# Autodesk Inventor assembly: SDS MK4i Swerve Module, NEOs
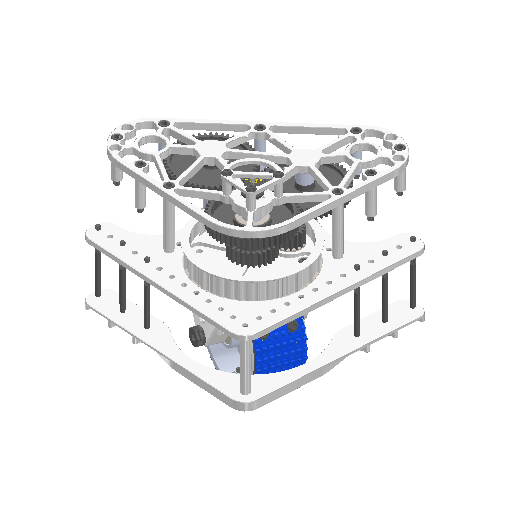
[picture p0: Inventor's stored thumbnail of the model, 512x512]
Saved by Autodesk Inventor 2023 (Build 270158000, 158)
## iProperties
Created: 2023-03-28
Part Number: SDS MK4i Swerve Module, NEOs
Document SubType Name: Assembly
Designer: jackc
Sending System: SOLIDWORKS 2021-2021301
MC: AMD64
MC_MODEL: Intel64 Family 6 Model 158 Stepping 10, GenuineIntel
OS: Windows_NT
FRU: Parasolid Version 32.1, build 255,  1- 1-2021
FORMAT: text
GUISE: transmit
KEY: SDS MK4i Swerve Module, NEOs
FILE: SDS MK4i Swerve Module, NEOs.x_t
DATE: Sun Dec  5 23:34:20 2021
Author: jackc
## Documents named in this file (54)
- J:\My Drive\1939\2_Design\2023-2024\Parts\Swerve\SDS MK4i Swerve Module, unpopulated.iam
- J:\My Drive\1939\2_Design\2023-2024\Parts\Swerve\Screw, 10-32 X .25, Button, 91255A261.ipt
- J:\My Drive\1939\2_Design\2023-2024\Parts\Swerve\Screw, Shoulder, .375 X 2.5, 5_16-18, 91259A634.ipt
- J:\My Drive\1939\2_Design\2023-2024\Parts\Swerve\Screw, .25-20 X 1 Socket, 91251A542.ipt
- J:\My Drive\1939\2_Design\2023-2024\Parts\Swerve\Screw, .25-20 X .625, 91251A539.ipt
- J:\My Drive\1939\2_Design\2023-2024\Parts\Swerve\Screw, 12-24 X .625, Flat, 91253A282.ipt
- J:\My Drive\1939\2_Design\2023-2024\Parts\Swerve\Screw, 10-32 X 1.375, 90044A202.ipt
- J:\My Drive\1939\2_Design\2023-2024\Parts\Swerve\Screw, 10-32 X 2.25, 91251A354.ipt
- J:\My Drive\1939\2_Design\2023-2024\Parts\Swerve\Screw, 8-32 X 2.5, 91251A207.ipt
- J:\My Drive\1939\2_Design\2023-2024\Parts\Swerve\Screw, 8-32 X .875, Button, 91255A166.ipt
- J:\My Drive\1939\2_Design\2023-2024\Parts\Swerve\Screw, 8-32 X .875, Button, 91255A166_1.ipt
- J:\My Drive\1939\2_Design\2023-2024\Parts\Swerve\Shim, 8mm ID X 14mm OD X .5mm Thick, 98055A115.ipt
- J:\My Drive\1939\2_Design\2023-2024\Parts\Swerve\Bearing, 6802.ipt
- J:\My Drive\1939\2_Design\2023-2024\Parts\Swerve\Bearing, R6ZZ.ipt
- J:\My Drive\1939\2_Design\2023-2024\Parts\Swerve\Bearing, R8ZZ.ipt
- J:\My Drive\1939\2_Design\2023-2024\Parts\Swerve\Bearing, 688.ipt
- J:\My Drive\1939\2_Design\2023-2024\Parts\Swerve\Bearing, .375 ThunderHex, Flanged, 217-5829.ipt
- J:\My Drive\1939\2_Design\2023-2024\Parts\Swerve\Bevel Gear, 1545.ipt
- J:\My Drive\1939\2_Design\2023-2024\Parts\Swerve\Bearing, R188ZZ, 217-3489.ipt
- J:\My Drive\1939\2_Design\2023-2024\Parts\Swerve\Bearing, A035XPO_SA035XPO.ipt
- J:\My Drive\1939\2_Design\2023-2024\Parts\Swerve\Double Gear, 20DP, 27T, 50T.ipt
- J:\My Drive\1939\2_Design\2023-2024\Parts\Swerve\Gear, 50T, 20DP, .375Hex.ipt
- J:\My Drive\1939\2_Design\2023-2024\Parts\Swerve\Bevel Gear, 4515.ipt
- J:\My Drive\1939\2_Design\2023-2024\Parts\Swerve\Gear, 20DP, 16T, .375Hex, 217-5451.ipt
- J:\My Drive\1939\2_Design\2023-2024\Parts\Swerve\MK4i Steering Shaft Tall(Default).ipt
- J:\My Drive\1939\2_Design\2023-2024\Parts\Swerve\MK4i Steering Shaft Tall(Default)_1.ipt
- J:\My Drive\1939\2_Design\2023-2024\Parts\Swerve\MK4i Steering Shaft Spacer.ipt
- J:\My Drive\1939\2_Design\2023-2024\Parts\Swerve\MK4 Intermediate Shaft(Default).ipt
- J:\My Drive\1939\2_Design\2023-2024\Parts\Swerve\MK3 Center Column(Default).ipt
- J:\My Drive\1939\2_Design\2023-2024\Parts\Swerve\MK4i Shaft, Drive Idler.ipt
- J:\My Drive\1939\2_Design\2023-2024\Parts\Swerve\CANcoder Assembly.iam
- J:\My Drive\1939\2_Design\2023-2024\Parts\Swerve\magnet.ipt
- J:\My Drive\1939\2_Design\2023-2024\Parts\Swerve\MK4i Master Part(NEO Config).ipt
- J:\My Drive\1939\2_Design\2023-2024\Parts\Swerve\MK4i Master Part(NEO Config)_1.ipt
- J:\My Drive\1939\2_Design\2023-2024\Parts\Swerve\MK4i Master Part(NEO Config)_2.ipt
- J:\My Drive\1939\2_Design\2023-2024\Parts\Swerve\MK4i Master Part(NEO Config)_3.ipt
- J:\My Drive\1939\2_Design\2023-2024\Parts\Swerve\MK4i Master Part(NEO Config)_4.ipt
- J:\My Drive\1939\2_Design\2023-2024\Parts\Swerve\MK4i Master Part(NEO Config)_5.ipt
- J:\My Drive\1939\2_Design\2023-2024\Parts\Swerve\MK4i Master Part(NEO Config)_6.ipt
- J:\My Drive\1939\2_Design\2023-2024\Parts\Swerve\MK4i Master Part(NEO Config)_7.ipt
- J:\My Drive\1939\2_Design\2023-2024\Parts\Swerve\MK4i Master Part(NEO Config)_8.ipt
- J:\My Drive\1939\2_Design\2023-2024\Parts\Swerve\MK4i Master Part(NEO Config)_9.ipt
- J:\My Drive\1939\2_Design\2023-2024\Parts\Swerve\MK4i Master Part(NEO Config)_10.ipt
- J:\My Drive\1939\2_Design\2023-2024\Parts\Swerve\MK4i Master Part(NEO Config)_11.ipt
- J:\My Drive\1939\2_Design\2023-2024\Parts\Swerve\MK4i Master Part(NEO Config)_12.ipt
- J:\My Drive\1939\2_Design\2023-2024\Parts\Swerve\MK4i Master Part(NEO Config)_13.ipt
- J:\My Drive\1939\2_Design\2023-2024\Parts\Swerve\MK4i Master Part(NEO Config)_14.ipt
- J:\My Drive\1939\2_Design\2023-2024\Parts\Swerve\MK4i Master Part(NEO Config)_15.ipt
- J:\My Drive\1939\2_Design\2023-2024\Parts\Swerve\MK4i Master Part(NEO Config)_16.ipt
- J:\My Drive\1939\2_Design\2023-2024\Parts\Swerve\MK4 Billet Wheel Assembly.iam
- J:\My Drive\1939\2_Design\2023-2024\Parts\Swerve\MK3 Base Pulley Tall.ipt
- J:\My Drive\1939\2_Design\2023-2024\Parts\Swerve\Wheel Mount A(Default).ipt
- J:\My Drive\1939\2_Design\2023-2024\Parts\Swerve\Wheel Mount B Gen2(Default).ipt
- J:\My Drive\1939\2_Design\2023-2024\Parts\Swerve\MK4 Wheel Spacer(Default).ipt
## Components (83 placed, 53 different names)
1. Double Gear, 20DP, 27T, 50T — Insert:20, Insert:23, Insert:27
2. Gear, 50T, 20DP, .375Hex — Insert:73
3. Gear, 50T, 20DP, .375Hex:1 — Insert:70, Insert:72
4. Bevel Gear, 4515 — Mate:16, Mate:17, Mate:18
5. Gear, 20DP, 16T, .375Hex, 217-5451 — Insert:21
6. MK4i Steering Shaft Tall(Default) — Insert:71, Insert:74, Insert:75
7. MK4i Steering Shaft Tall(Default)_1 — Insert:72, Insert:74
8. MK4i Steering Shaft Spacer — Insert:70, Insert:76
9. MK4 Intermediate Shaft(Default) — Insert:3, Insert:4, Insert:5, Insert:21, Insert:22
10. MK3 Center Column(Default) — Mate:13, Mate:14, Insert:28, Insert:78
11. MK4i Shaft, Drive Idler — Insert:17
12. CANcoder Assembly [sub-assembly]
13. magnet — Insert:28
14. MK4i Master Part(NEO Config) — Insert:54
15. MK4i Master Part(NEO Config)_1 — Insert:51, Insert:52
16. MK4i Master Part(NEO Config)_2 — Insert:8, Insert:9
17. MK4i Master Part(NEO Config)_3 — Insert:66
18. MK4i Master Part(NEO Config)_4 — Insert:64
19. MK4i Master Part(NEO Config)_5 — Insert:69
20. MK4i Master Part(NEO Config)_6 — Insert:67
21. MK4i Master Part(NEO Config)_7 — Insert:6, Insert:7
22. MK4i Master Part(NEO Config)_8 — Mate:24, Insert:49
23. MK4i Master Part(NEO Config)_9 — Insert:37
24. MK4i Master Part(NEO Config)_10 — Insert:38, Insert:48
25. MK4i Master Part(NEO Config)_11 — Insert:37, Insert:38, Mate:24, Insert:45, Insert:46, Insert:47
26. MK4i Master Part(NEO Config)_12 — Insert:6, Mate:10, Insert:32, Insert:33, Mate:19, Mate:20, Mate:22, Insert:43, Insert:44, Mate:45
27. MK4i Master Part(NEO Config)_13 — Insert:9, Insert:34, Insert:48, Insert:49, Insert:50, Insert:51, Insert:53, Insert:54, Insert:58, Insert:59, Insert:60, Insert:61, Insert:62, Insert:63, Insert:64, Insert:65, Insert:66, Insert:67, Insert:68, Insert:69, Mate:28, Insert:77, Insert:79
28. MK4i Master Part(NEO Config)_14 — Mate:9, Insert:7, Insert:8, Insert:33, Insert:52, Insert:55, Insert:56, Insert:57, Mate:25, Mate:26, Mate:27, Mate:40, Mate:41, Mate:42, Mate:43, Mate:44
29. MK4i Master Part(NEO Config)_15 — Insert:68
30. MK4i Master Part(NEO Config)_16 — Insert:65
31. MK4 Billet Wheel Assembly [sub-assembly] — Mate:3, Insert:29, Mate:16, Mate:17, Mate:18
32. MK3 Base Pulley Tall — Insert:1, Insert:2, Insert:10, Insert:11, Insert:13, Insert:15, Mate:13, Mate:14, Insert:16, Insert:23, Insert:24
33. Wheel Mount A(Default) — Mate:2, Mate:5, Insert:2, Insert:24, Insert:25
34. Wheel Mount B Gen2(Default) — Insert:1, Insert:12, Insert:15, Insert:31
35. MK4 Wheel Spacer(Default) — Insert:30, Insert:31
36. Bearing, A035XPO_SA035XPO — Insert:55
37. Bearing, 688:3 — Insert:73, Mate:28
38. Bearing, 688:2 — Insert:76, Insert:77
39. Bearing, R188ZZ, 217-3489 — Insert:71, Insert:75
40. Bearing, 688:1 — Mate:9, Insert:17
41. Bevel Gear, 1545 — Insert:4
42. Bearing, .375 ThunderHex, Flanged, 217-5829 — Insert:13
43. Bearing, 688 — Insert:5, Insert:12
44. Bearing, R8ZZ — Insert:29, Insert:30
45. Bearing, R6ZZ — Mate:3
46. Bearing, 6802:2 — Insert:20
47. Bearing, 6802:1 — Insert:78, Insert:79
48. Bearing, 6802 — Insert:27
49. Screw, 10-32 X .25, Button, 91255A261 — Mate:26
50. Screw, 10-32 X .25, Button, 91255A261:1 — Mate:27
51. Screw, 10-32 X .25, Button, 91255A261:2 — Mate:25, Mate:44
52. Screw, 10-32 X .25, Button, 91255A261:3 — Insert:56
53. Screw, 10-32 X .25, Button, 91255A261:4 — Insert:57
54. Screw, Shoulder, .375 X 2.5, 5_16-18, 91259A634 — Insert:25
55. Screw, .25-20 X 1 Socket, 91251A542 — Mate:2
56. Screw, .25-20 X 1 Socket, 91251A542:1 — Mate:5
57. Screw, .25-20 X .625, 91251A539 — Insert:10
58. Screw, .25-20 X .625, 91251A539:1 — Insert:11
59. Screw, .25-20 X .625, 91251A539:2 — Insert:16
60. Screw, 12-24 X .625, Flat, 91253A282 — Insert:22
61. Screw, 10-32 X 1.375, 90044A202 — Insert:58
62. Screw, 10-32 X 1.375, 90044A202:1 — Insert:60
63. Screw, 10-32 X 1.375, 90044A202:2 — Insert:63
64. Screw, 10-32 X 1.375, 90044A202:3 — Insert:62
65. Screw, 10-32 X 1.375, 90044A202:4 — Insert:59
66. Screw, 10-32 X 1.375, 90044A202:5 — Insert:61
67. Screw, 10-32 X 2.25, 91251A354 — Insert:53
68. Screw, 10-32 X 2.25, 91251A354:1 — Insert:50
69. Screw, 10-32 X 2.25, 91251A354:2 — Insert:34
70. Screw, 10-32 X 2.25, 91251A354:3 — Insert:44
71. Screw, 8-32 X 2.5, 91251A207 — Mate:10, Mate:42
72. Screw, 8-32 X 2.5, 91251A207:1 — Mate:22, Mate:43
73. Screw, 8-32 X 2.5, 91251A207:2 — Insert:43
74. Screw, 8-32 X 2.5, 91251A207:3 — Mate:20, Mate:41
75. Screw, 8-32 X 2.5, 91251A207:4 — Mate:19, Mate:40
76. Screw, 8-32 X 2.5, 91251A207:5 — Insert:32
77. Screw, 8-32 X .875, Button, 91255A166 — Insert:36, Insert:47
78. Screw, 8-32 X .875, Button, 91255A166_1 — Insert:36
79. Screw, 8-32 X .875, Button, 91255A166:1 — Insert:35, Insert:45
80. Screw, 8-32 X .875, Button, 91255A166_1:1 — Insert:35
81. Screw, 8-32 X .875, Button, 91255A166:2 — Mate:23, Insert:46
82. Screw, 8-32 X .875, Button, 91255A166_1:2 — Mate:23
83. Shim, 8mm ID X 14mm OD X .5mm Thick, 98055A115 — Insert:3
## Relationships (96: Insert 71, Mate 25)
- Mate:2: Wheel Mount A(Default) ↔ Screw, .25-20 X 1 Socket, 91251A542
- Mate:3: MK4 Billet Wheel Assembly ↔ Bearing, R6ZZ
- Mate:5: Wheel Mount A(Default) ↔ Screw, .25-20 X 1 Socket, 91251A542:1
- Insert:1: MK3 Base Pulley Tall ↔ Wheel Mount B Gen2(Default)
- Insert:2: MK3 Base Pulley Tall ↔ Wheel Mount A(Default)
- Insert:3 (0.404 mm): MK4 Intermediate Shaft(Default) ↔ Shim, 8mm ID X 14mm OD X .5mm Thick, 98055A115
- Insert:4: MK4 Intermediate Shaft(Default) ↔ Bevel Gear, 1545
- Insert:5: MK4 Intermediate Shaft(Default) ↔ Bearing, 688
- Mate:9: MK4i Master Part(NEO Config)_14 ↔ Bearing, 688:1
- Insert:6: MK4i Master Part(NEO Config)_7 ↔ MK4i Master Part(NEO Config)_12
- Insert:7: MK4i Master Part(NEO Config)_7 ↔ MK4i Master Part(NEO Config)_14
- Mate:10: MK4i Master Part(NEO Config)_12 ↔ Screw, 8-32 X 2.5, 91251A207
- Insert:8: MK4i Master Part(NEO Config)_2 ↔ MK4i Master Part(NEO Config)_14
- Insert:9: MK4i Master Part(NEO Config)_2 ↔ MK4i Master Part(NEO Config)_13
- Insert:10: MK3 Base Pulley Tall ↔ Screw, .25-20 X .625, 91251A539
- Insert:11: MK3 Base Pulley Tall ↔ Screw, .25-20 X .625, 91251A539:1
- Insert:12: Wheel Mount B Gen2(Default) ↔ Bearing, 688
- Insert:13: MK3 Base Pulley Tall ↔ Bearing, .375 ThunderHex, Flanged, 217-5829
- Insert:15: MK3 Base Pulley Tall ↔ Wheel Mount B Gen2(Default)
- Mate:13: MK3 Center Column(Default) ↔ MK3 Base Pulley Tall
- Mate:14: MK3 Center Column(Default) ↔ MK3 Base Pulley Tall
- Insert:16: MK3 Base Pulley Tall ↔ Screw, .25-20 X .625, 91251A539:2
- Insert:17: MK4i Shaft, Drive Idler ↔ Bearing, 688:1
- Insert:20: Double Gear, 20DP, 27T, 50T ↔ Bearing, 6802:2
- Insert:21 (-2 mm): Gear, 20DP, 16T, .375Hex, 217-5451 ↔ MK4 Intermediate Shaft(Default)
- Insert:22 (-2.5 mm): MK4 Intermediate Shaft(Default) ↔ Screw, 12-24 X .625, Flat, 91253A282
- Insert:23: Double Gear, 20DP, 27T, 50T ↔ MK3 Base Pulley Tall
- Insert:24: MK3 Base Pulley Tall ↔ Wheel Mount A(Default)
- Insert:25: Wheel Mount A(Default) ↔ Screw, Shoulder, .375 X 2.5, 5_16-18, 91259A634
- Insert:27: Double Gear, 20DP, 27T, 50T ↔ Bearing, 6802
- Insert:28: MK3 Center Column(Default) ↔ magnet
- Insert:29: MK4 Billet Wheel Assembly ↔ Bearing, R8ZZ
- Insert:30: MK4 Wheel Spacer(Default) ↔ Bearing, R8ZZ
- Insert:31: Wheel Mount B Gen2(Default) ↔ MK4 Wheel Spacer(Default)
- Mate:16: Bevel Gear, 4515 ↔ MK4 Billet Wheel Assembly
- Mate:17: Bevel Gear, 4515 ↔ MK4 Billet Wheel Assembly
- Mate:18: Bevel Gear, 4515 ↔ MK4 Billet Wheel Assembly
- Insert:32: MK4i Master Part(NEO Config)_12 ↔ Screw, 8-32 X 2.5, 91251A207:5
- Insert:33 (50.8 mm): MK4i Master Part(NEO Config)_12 ↔ MK4i Master Part(NEO Config)_14
- Mate:19: MK4i Master Part(NEO Config)_12 ↔ Screw, 8-32 X 2.5, 91251A207:4
- Mate:20: MK4i Master Part(NEO Config)_12 ↔ Screw, 8-32 X 2.5, 91251A207:3
- Mate:22: MK4i Master Part(NEO Config)_12 ↔ Screw, 8-32 X 2.5, 91251A207:1
- Insert:34: MK4i Master Part(NEO Config)_13 ↔ Screw, 10-32 X 2.25, 91251A354:2
- Insert:35: Screw, 8-32 X .875, Button, 91255A166:1 ↔ Screw, 8-32 X .875, Button, 91255A166_1:1
- Insert:36: Screw, 8-32 X .875, Button, 91255A166 ↔ Screw, 8-32 X .875, Button, 91255A166_1
- Mate:23: Screw, 8-32 X .875, Button, 91255A166:2 ↔ Screw, 8-32 X .875, Button, 91255A166_1:2
- Insert:37: MK4i Master Part(NEO Config)_9 ↔ MK4i Master Part(NEO Config)_11
- Insert:38: MK4i Master Part(NEO Config)_10 ↔ MK4i Master Part(NEO Config)_11
- Mate:24: MK4i Master Part(NEO Config)_8 ↔ MK4i Master Part(NEO Config)_11
- Insert:43: MK4i Master Part(NEO Config)_12 ↔ Screw, 8-32 X 2.5, 91251A207:2
- Insert:44: MK4i Master Part(NEO Config)_12 ↔ Screw, 10-32 X 2.25, 91251A354:3
- Insert:45: MK4i Master Part(NEO Config)_11 ↔ Screw, 8-32 X .875, Button, 91255A166:1
- Insert:46: MK4i Master Part(NEO Config)_11 ↔ Screw, 8-32 X .875, Button, 91255A166:2
- Insert:47: MK4i Master Part(NEO Config)_11 ↔ Screw, 8-32 X .875, Button, 91255A166
- Insert:48: MK4i Master Part(NEO Config)_10 ↔ MK4i Master Part(NEO Config)_13
- Insert:49: MK4i Master Part(NEO Config)_8 ↔ MK4i Master Part(NEO Config)_13
- Insert:50: MK4i Master Part(NEO Config)_13 ↔ Screw, 10-32 X 2.25, 91251A354:1
- Insert:51: MK4i Master Part(NEO Config)_1 ↔ MK4i Master Part(NEO Config)_13
- Insert:52: MK4i Master Part(NEO Config)_1 ↔ MK4i Master Part(NEO Config)_14
- Insert:53: MK4i Master Part(NEO Config)_13 ↔ Screw, 10-32 X 2.25, 91251A354
- Insert:54: MK4i Master Part(NEO Config) ↔ MK4i Master Part(NEO Config)_13
- Insert:55: MK4i Master Part(NEO Config)_14 ↔ Bearing, A035XPO_SA035XPO
- Insert:56: MK4i Master Part(NEO Config)_14 ↔ Screw, 10-32 X .25, Button, 91255A261:3
- Insert:57: MK4i Master Part(NEO Config)_14 ↔ Screw, 10-32 X .25, Button, 91255A261:4
- Mate:25: MK4i Master Part(NEO Config)_14 ↔ Screw, 10-32 X .25, Button, 91255A261:2
- Mate:26: MK4i Master Part(NEO Config)_14 ↔ Screw, 10-32 X .25, Button, 91255A261
- Mate:27: MK4i Master Part(NEO Config)_14 ↔ Screw, 10-32 X .25, Button, 91255A261:1
- Insert:58: MK4i Master Part(NEO Config)_13 ↔ Screw, 10-32 X 1.375, 90044A202
- Insert:59: MK4i Master Part(NEO Config)_13 ↔ Screw, 10-32 X 1.375, 90044A202:4
- Insert:60: MK4i Master Part(NEO Config)_13 ↔ Screw, 10-32 X 1.375, 90044A202:1
- Insert:61: MK4i Master Part(NEO Config)_13 ↔ Screw, 10-32 X 1.375, 90044A202:5
- Insert:62: MK4i Master Part(NEO Config)_13 ↔ Screw, 10-32 X 1.375, 90044A202:3
- Insert:63: MK4i Master Part(NEO Config)_13 ↔ Screw, 10-32 X 1.375, 90044A202:2
- Insert:64: MK4i Master Part(NEO Config)_4 ↔ MK4i Master Part(NEO Config)_13
- Insert:65: MK4i Master Part(NEO Config)_13 ↔ MK4i Master Part(NEO Config)_16
- Insert:66: MK4i Master Part(NEO Config)_3 ↔ MK4i Master Part(NEO Config)_13
- Insert:67: MK4i Master Part(NEO Config)_6 ↔ MK4i Master Part(NEO Config)_13
- Insert:68: MK4i Master Part(NEO Config)_13 ↔ MK4i Master Part(NEO Config)_15
- Insert:69: MK4i Master Part(NEO Config)_5 ↔ MK4i Master Part(NEO Config)_13
- Insert:70: Gear, 50T, 20DP, .375Hex:1 ↔ MK4i Steering Shaft Spacer
- Insert:71: MK4i Steering Shaft Tall(Default) ↔ Bearing, R188ZZ, 217-3489
- Insert:72: Gear, 50T, 20DP, .375Hex:1 ↔ MK4i Steering Shaft Tall(Default)_1
- Insert:73 (0.127 mm): Gear, 50T, 20DP, .375Hex ↔ Bearing, 688:3
- Mate:28: MK4i Master Part(NEO Config)_13 ↔ Bearing, 688:3
- Insert:74: MK4i Steering Shaft Tall(Default) ↔ MK4i Steering Shaft Tall(Default)_1
- Insert:75: MK4i Steering Shaft Tall(Default) ↔ Bearing, R188ZZ, 217-3489
- Insert:76: MK4i Steering Shaft Spacer ↔ Bearing, 688:2
- Insert:77: MK4i Master Part(NEO Config)_13 ↔ Bearing, 688:2
- Insert:78: MK3 Center Column(Default) ↔ Bearing, 6802:1
- Insert:79 (-1 mm): MK4i Master Part(NEO Config)_13 ↔ Bearing, 6802:1
- Mate:40: MK4i Master Part(NEO Config)_14 ↔ Screw, 8-32 X 2.5, 91251A207:4
- Mate:41: MK4i Master Part(NEO Config)_14 ↔ Screw, 8-32 X 2.5, 91251A207:3
- Mate:42: MK4i Master Part(NEO Config)_14 ↔ Screw, 8-32 X 2.5, 91251A207
- Mate:43: MK4i Master Part(NEO Config)_14 ↔ Screw, 8-32 X 2.5, 91251A207:1
- Mate:44: MK4i Master Part(NEO Config)_14 ↔ Screw, 10-32 X .25, Button, 91255A261:2
- Mate:45: MK4i Master Part(NEO Config)_12
